# Autodesk Inventor assembly: 23-010
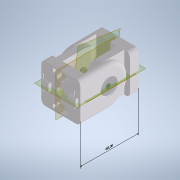
[picture p0: Inventor's stored thumbnail of the model, 180x180]
Saved by Autodesk Inventor 2022 (Build 260153000, 153)
## iProperties
Created: 2004-10-21
Part Number: 23-010
Document SubType Name: Assembly
Designer: Chapin
Manufacturer: Standard
Standards Organization: Custom
Mass: 167.294 g
Surface Area: 304.477 cm^2
Volume: 58.9179 cm^3
Density: 2.83944 g/cm^3
Author: Chapin
## Documents named in this file (6)
- C:\Users\matte\Documents\GitHub\MDM-CyberOrto-CAD\Parker components\05-Handles_Hinges\13-Pivot Joints\23-010.iam
- C:\Users\matte\Documents\GitHub\MDM-CyberOrto-CAD\Parker components\05-Handles_Hinges\13-Pivot Joints\23-010Z1.ipt
- C:\Users\matte\Documents\GitHub\MDM-CyberOrto-CAD\Parker components\05-Handles_Hinges\13-Pivot Joints\23-010Z2.ipt
- C:\Users\matte\Documents\GitHub\MDM-CyberOrto-CAD\Parker components\05-Handles_Hinges\13-Pivot Joints\23-010Z3.ipt
- C:\Users\matte\Documents\GitHub\MDM-CyberOrto-CAD\Parker components\05-Handles_Hinges\13-Pivot Joints\23-010Z4.ipt
- C:\Users\matte\Documents\GitHub\MDM-CyberOrto-CAD\Parker components\05-Handles_Hinges\13-Pivot Joints\24-212-8.ipt
## Components (12 placed, 5 different names)
1. 23-010Z1:1 — Mate:3, Mate:4, Mate:7, Mate:8, Mate:9, Mate:10, Mate:11, Mate:12, Mate:13, Mate:14, Mate:15, Mate:16, Angle:1, Mate:23, Mate:26, Mate:30, Angle:4, Angle:5
2. 23-010Z1:2 — Mate:1, Mate:2, Mate:5, Mate:6, Mate:10, Mate:17, Mate:18, Mate:19, Mate:20, Mate:21, Mate:22, Angle:1, Mate:24, Mate:25, Mate:27, Angle:2, Angle:3
3. 23-010Z2:1 — Mate:20, Mate:21, Mate:22
4. 23-010Z2:2 — Mate:17, Mate:18, Mate:19
5. 23-010Z2:3 — Mate:14, Mate:15, Mate:16
6. 23-010Z2:4 — Mate:11, Mate:12, Mate:13
7. 23-010Z3:1 — Mate:1, Mate:2
8. 23-010Z3:2 — Mate:3, Mate:4
9. 23-010Z4:1 — Mate:7, Mate:8
10. 23-010Z4:2 — Mate:5, Mate:6, Mate:9
11. 24-212-8:1 — Mate:23, Mate:24
12. 24-212-8:2 — Mate:25, Mate:26
## Relationships (38: Mate 32, Angle 6)
- Mate:1: 23-010Z1:2 ↔ 23-010Z3:1
- Mate:2: 23-010Z1:2 ↔ 23-010Z3:1
- Mate:3: 23-010Z1:1 ↔ 23-010Z3:2
- Mate:4: 23-010Z1:1 ↔ 23-010Z3:2
- Mate:5: 23-010Z1:2 ↔ 23-010Z4:2
- Mate:6: 23-010Z1:2 ↔ 23-010Z4:2
- Mate:7: 23-010Z1:1 ↔ 23-010Z4:1
- Mate:8: 23-010Z1:1 ↔ 23-010Z4:1
- Mate:9: 23-010Z1:1 ↔ 23-010Z4:2
- Mate:10: 23-010Z1:1 ↔ 23-010Z1:2
- Mate:11: 23-010Z1:1 ↔ 23-010Z2:4
- Mate:12 (0.17 mm): 23-010Z1:1 ↔ 23-010Z2:4
- Mate:13 (0.19 mm): 23-010Z1:1 ↔ 23-010Z2:4
- Mate:14: 23-010Z1:1 ↔ 23-010Z2:3
- Mate:15 (0.17 mm): 23-010Z1:1 ↔ 23-010Z2:3
- Mate:16 (0.19 mm): 23-010Z1:1 ↔ 23-010Z2:3
- Mate:17: 23-010Z1:2 ↔ 23-010Z2:2
- Mate:18 (0.17 mm): 23-010Z1:2 ↔ 23-010Z2:2
- Mate:19 (0.19 mm): 23-010Z1:2 ↔ 23-010Z2:2
- Mate:20 (0.19 mm): 23-010Z1:2 ↔ 23-010Z2:1
- Mate:21: 23-010Z1:2 ↔ 23-010Z2:1
- Mate:22 (0.17 mm): 23-010Z1:2 ↔ 23-010Z2:1
- Angle:1 (270 deg): 23-010Z1:1 ↔ 23-010Z1:2
- Mate:23: 23-010Z1:1 ↔ 24-212-8:1
- Mate:24 (-1 mm): 23-010Z1:2 ↔ 24-212-8:1
- Mate:25: 23-010Z1:2 ↔ 24-212-8:2
- Mate:26 (-1 mm): 23-010Z1:1 ↔ 24-212-8:2
- Mate:27: 23-010Z1:2
- Mate:28
- Angle:2 (90 deg): 23-010Z1:2
- Mate:29
- Angle:3 (90 deg): 23-010Z1:2
- Mate:30: 23-010Z1:1
- Mate:31
- Angle:4 (90 deg): 23-010Z1:1
- Mate:32
- Angle:5 (90 deg): 23-010Z1:1
- Angolo:6 [Angle] (0 deg)
